# Autodesk Inventor assembly: Cryostat Installation - Working Copy
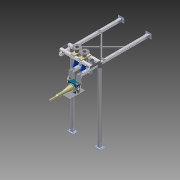
[picture p0: Inventor's stored thumbnail of the model, 180x180]
Saved by Autodesk Inventor 2015 (Build 190159000, 159)
## iProperties
Created: 2012-10-02
Part Number: Cryostat Installation - Working Copy
Document SubType Name: Assembly
Designer: Gary
Author: Gary
## Documents named in this file (10)
- C:\Users\Brogan Thomas\Documents\GitHub\Fridge_drawing\Fridge_drawing.iam
- C:\Users\Brogan Thomas\Documents\Inventor\HIFROST\HIFROSTCad\Cryostat Support - Main Frame.iam
- C:\Users\Brogan Thomas\Documents\Inventor\HIFROST\HIFROSTCad\Deck for LHe Dewar.iam
- C:\Users\Brogan Thomas\Documents\Inventor\HIFROST\HIFROSTCad\Cryostat w Mount in BL.iam
- C:\Users\Brogan Thomas\Documents\Inventor\HIFROST\HIFROSTCad\72-110-30.iam
- C:\Users\Brogan Thomas\Documents\Inventor\HIFROST\HIFROSTCad\72-110-40.iam
- C:\Users\Brogan Thomas\Documents\Inventor\HIFROST\HIFROSTCad\HIFROST RF Assy.iam
- C:\Users\Brogan Thomas\Documents\Inventor\HIFROST\HIFROSTCad\EIO Support Arm.iam
- C:\Users\Brogan Thomas\Documents\Inventor\HIFROST\HIFROSTCad\Fridge Flange Plate Nut.ipt
- C:\Users\Brogan Thomas\Documents\Inventor\HIFROST\Imported Components\90293A439\90293A439.ipt
## Components (10 placed, 9 different names)
1. Cryostat Support - Main Frame:1 [sub-assembly] — Flush:8, Flush:9, Mate:10, Mate:11
2. Deck for LHe Dewar:1 [sub-assembly] — Flush:7, Flush:8, Flush:9
3. Cryostat w Mount in BL:1 [sub-assembly] — Mate:4, Mate:5, Mate:6, Insert:1, Flush:10, Mate:12, Mate:13, Mate:14, Mate:15
4. 72-110-30:1 [sub-assembly] — Mate:4, Mate:5, Mate:6, Mate:7, Mate:8, Mate:9
5. 72-110-40:1 [sub-assembly] — Mate:7, Mate:8, Mate:9
6. HIFROST RF Assy:1 [sub-assembly] — Insert:1, Angle:2
7. EIO Support Arm:1 [sub-assembly] — Mate:10, Mate:11
8. Fridge Flange Plate Nut:1 — Flush:10
9. 90293A439:1 — Mate:12, Mate:14
10. 90293A439:2 — Mate:13, Mate:15
## Relationships (24: Mate 15, Flush 6, Angle 2, Insert 1)
- [Flush]: Cryostat w Mount in BL:1
- [Mate]: Cryostat w Mount in BL:1
- [Mate]: Cryostat w Mount in BL:1
- [Angle] (0 deg): Cryostat w Mount in BL:1
- [Mate] (12.7 mm): Cryostat Support - Main Frame:1 ↔ Cryostat w Mount in BL:1
- [Flush] (6.35 mm): Cryostat Support - Main Frame:1 ↔ Cryostat w Mount in BL:1
- Flush:7: Deck for LHe Dewar:1
- Flush:8 (-482.6 mm): Cryostat Support - Main Frame:1 ↔ Deck for LHe Dewar:1
- Flush:9: Cryostat Support - Main Frame:1 ↔ Deck for LHe Dewar:1
- Mate:4: Cryostat w Mount in BL:1 ↔ 72-110-30:1
- Mate:5: Cryostat w Mount in BL:1 ↔ 72-110-30:1
- Mate:6: Cryostat w Mount in BL:1 ↔ 72-110-30:1
- Mate:7: 72-110-30:1 ↔ 72-110-40:1
- Mate:8: 72-110-30:1 ↔ 72-110-40:1
- Mate:9: 72-110-30:1 ↔ 72-110-40:1
- Insert:1: Cryostat w Mount in BL:1 ↔ HIFROST RF Assy:1
- Angle:2 (180 deg): HIFROST RF Assy:1
- Mate:10: Cryostat Support - Main Frame:1 ↔ EIO Support Arm:1
- Mate:11: Cryostat Support - Main Frame:1 ↔ EIO Support Arm:1
- Flush:10: Cryostat w Mount in BL:1 ↔ Fridge Flange Plate Nut:1
- Mate:12: Cryostat w Mount in BL:1 ↔ 90293A439:1
- Mate:13: Cryostat w Mount in BL:1 ↔ 90293A439:2
- Mate:14: Cryostat w Mount in BL:1 ↔ 90293A439:1
- Mate:15: Cryostat w Mount in BL:1 ↔ 90293A439:2
